# Autodesk Inventor assembly: build
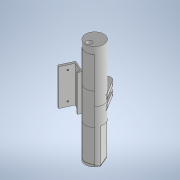
[picture p0: Inventor's stored thumbnail of the model, 180x180]
Saved by Autodesk Inventor 2020 (Build 240168000, 168)
## iProperties
Created: 2022-10-25
Part Number: build
Document SubType Name: Assembly
Designer: zigma
Author: zigma
## Documents named in this file (7)
- C:\Users\zigma\Documents\Work\desktop lamp\DesktopRGBLamp\Design\build.iam
- C:\Users\zigma\Documents\Work\desktop lamp\DesktopRGBLamp\Design\body_cover.ipt
- C:\Users\zigma\Documents\Work\desktop lamp\DesktopRGBLamp\Design\body_part1.ipt
- C:\Users\zigma\Documents\Work\desktop lamp\DesktopRGBLamp\Design\body_part2.ipt
- C:\Users\zigma\Documents\Work\desktop lamp\DesktopRGBLamp\Design\bracket.ipt
- C:\Users\zigma\Documents\Work\desktop lamp\DesktopRGBLamp\Design\holder.ipt
- C:\Users\zigma\Documents\Work\desktop lamp\DesktopRGBLamp\Design\lens.ipt
## Components (9 placed, 6 different names)
1. body_cover:1 — Жесткий:1
2. body_part1:1 — Жесткий:1, Жесткий:2, Жесткий:4
3. body_part2:1 — Жесткий:3, Жесткий:4, Жесткий:7
4. bracket:1 — Жесткий:3, С поворотом:1
5. holder:1 — С поворотом:1
6. lens:1 — Жесткий:6
7. bracket:2 — Жесткий:2
8. lens:2 — Жесткий:5, Жесткий:7
9. lens:3 — Жесткий:5, Жесткий:6
## Relationships (8: WeldJoint 7, RevoluteJoint 1)
- Жесткий:1 [WeldJoint]: body_cover:1 ↔ body_part1:1
- Жесткий:2 [WeldJoint]: body_part1:1 ↔ bracket:2
- Жесткий:3 [WeldJoint]: body_part2:1 ↔ bracket:1
- Жесткий:4 [WeldJoint]: body_part1:1 ↔ body_part2:1
- Жесткий:5 [WeldJoint]: lens:2 ↔ lens:3
- Жесткий:6 [WeldJoint]: lens:1 ↔ lens:3
- Жесткий:7 [WeldJoint]: body_part2:1 ↔ lens:2
- С поворотом:1 [RevoluteJoint]: bracket:1 ↔ holder:1
